# Autodesk Inventor assembly: zespolokno
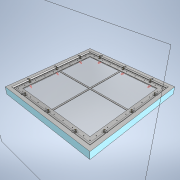
[picture p0: Inventor's stored thumbnail of the model, 180x180]
Saved by Autodesk Inventor 2021 (Build 250183000, 183)
## iProperties
Created: 2021-06-22
Part Number: zespolokno
Document SubType Name: Assembly
Designer: Wojciech Wołczek
Mass: 5787.78 g
Surface Area: 15277.7 cm^2
Volume: 11241.1 cm^3
Density: 0.514875 g/cm^3
Author: Wojciech Wołczek
## Documents named in this file (6)
- D:\OneDrive\Documents\autodesk\oknoadvanced\zespolokno.iam
- D:\OneDrive\Documents\autodesk\oknoadvanced\rama.ipt
- D:\OneDrive\Documents\autodesk\oknoadvanced\alu.ipt
- D:\OneDrive\Documents\autodesk\uchwytokno\zespoluchwyt.iam
- D:\OneDrive\Documents\autodesk\uchwytokno\krys.ipt
- D:\OneDrive\Documents\autodesk\oknoadvanced\glas.ipt
## Components (17 placed, 5 different names)
1. rama:1 — Zestawiające:1, Zestawiające:2, Zestawiające:3, Zestawiające:4, Zestawiające:5
2. alu:1 — Zestawiające:1, Zestawiające:2, Zestawiające:3, Zestawiające:4, Zestawiające:5, Zestawiające:6, Zestawiające:7, Zestawiające:8, Zestawiające:9, Zestawiające:10, Równoległe:3, Równoległe:4
3. krys:1 — Równoległe:1, Równoległe:2, Zestawiające:11
4. glas:1 — Równoległe:3, Równoległe:4, Równoległe:5, Równoległe:6
5. glas:2 — Zestawiające:11, Równoległe:5, Równoległe:6
6. zespoluchwyt:1 [sub-assembly] — Zestawiające:6, Zestawiające:7
7. zespoluchwyt:2 [sub-assembly]
8. zespoluchwyt:3 [sub-assembly]
9. zespoluchwyt:4 [sub-assembly]
10. zespoluchwyt:5 [sub-assembly]
11. zespoluchwyt:6 [sub-assembly]
12. zespoluchwyt:7 [sub-assembly]
13. zespoluchwyt:8 [sub-assembly]
14. zespoluchwyt:9 [sub-assembly]
15. zespoluchwyt:10 [sub-assembly]
16. zespoluchwyt:11 [sub-assembly]
17. zespoluchwyt:12 [sub-assembly]
## Component patterns: (4 elements), (3 elements, first: zespoluchwyt:1), Szyk komponentów 1:2 (3 elements), Szyk komponentów 1:3 (3 elements), Szyk komponentów 1:4 (3 elements)
## Relationships (17: Mate 11, Flush 6)
- Zestawiające:1 [Mate]: rama:1 ↔ alu:1
- Zestawiające:2 [Mate]: rama:1 ↔ alu:1
- Zestawiające:3 [Mate]: rama:1 ↔ alu:1
- Zestawiające:4 [Mate]: rama:1 ↔ alu:1
- Zestawiające:5 [Mate]: rama:1 ↔ alu:1
- Zestawiające:6 [Mate]: alu:1 ↔ zespoluchwyt:1
- Zestawiające:7 [Mate]: alu:1 ↔ zespoluchwyt:1
- Zestawiające:8 [Mate]: alu:1
- Zestawiające:9 [Mate]: alu:1
- Zestawiające:10 [Mate]: alu:1
- Równoległe:1 [Flush]: krys:1
- Równoległe:2 [Flush]: krys:1
- Równoległe:3 [Flush]: alu:1 ↔ glas:1
- Równoległe:4 [Flush]: alu:1 ↔ glas:1
- Zestawiające:11 [Mate]: krys:1 ↔ glas:2
- Równoległe:5 [Flush]: glas:1 ↔ glas:2
- Równoległe:6 [Flush]: glas:1 ↔ glas:2
